# Autodesk Inventor assembly: gear_set
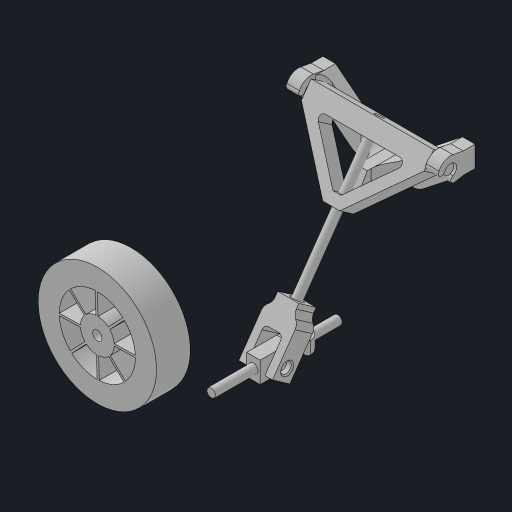
[picture p0: Inventor's stored thumbnail of the model, 512x512]
Saved by Autodesk Inventor 2023 (Build 270158000, 158)
## iProperties
Created: 2022-06-15
Part Number: gear_set
Document SubType Name: Assembly
Designer: legot
Author: legot
## Documents named in this file (8)
- C:\Users\legot\OneDrive\ドキュメント\Inventor\HIKOSAPO\Gear\gear_set.iam
- C:\Users\legot\OneDrive\ドキュメント\Inventor\HIKOSAPO\Gear\gear_connecotr1.ipt
- C:\Users\legot\OneDrive\ドキュメント\Inventor\HIKOSAPO\Gear\gear_connector2.ipt
- C:\Users\legot\OneDrive\ドキュメント\Inventor\HIKOSAPO\Gear\gear_shaft.ipt
- C:\Users\legot\OneDrive\ドキュメント\Inventor\HIKOSAPO\public_parts\Wheel_Φ50.ipt
- C:\Users\legot\OneDrive\ドキュメント\Inventor\HIKOSAPO\Gear\gear_rod.ipt
- C:\Users\legot\OneDrive\ドキュメント\Inventor\HIKOSAPO\Gear\gear_base1.ipt
- C:\Users\legot\OneDrive\ドキュメント\Inventor\HIKOSAPO\Gear\gear_base2.ipt
## Components (7 placed, 7 different names)
1. gear_connecotr1:1 — メイト:3, 挿入:1
2. gear_connector2:1 — メイト:2, メイト:3, 挿入:2
3. gear_shaft:1 — 挿入:1, メイト:4
4. Wheel_Φ50:1 — メイト:4
5. gear_rod:1 — 挿入:2, 挿入:3, 角度:2
6. gear_base1:1 — 挿入:3, メイト:5
7. gear_base2:1 — メイト:5, 角度:1, フラッシュ:1
## Relationships (10: Mate 4, Insert 3, Angle 2, Flush 1)
- メイト:2 [Mate]: gear_connector2:1
- メイト:3 [Mate]: gear_connecotr1:1 ↔ gear_connector2:1
- 挿入:1 [Insert] (-10 mm): gear_connecotr1:1 ↔ gear_shaft:1
- メイト:4 [Mate]: gear_shaft:1 ↔ Wheel_Φ50:1
- 挿入:2 [Insert]: gear_connector2:1 ↔ gear_rod:1
- 挿入:3 [Insert]: gear_rod:1 ↔ gear_base1:1
- メイト:5 [Mate]: gear_base1:1 ↔ gear_base2:1
- 角度:1 [Angle] (180 deg): gear_base2:1
- フラッシュ:1 [Flush]: gear_base2:1
- 角度:2 [Angle] (0 deg): gear_rod:1
